# Autodesk Inventor assembly: 176-DP(D-229)(F,D-231-1)
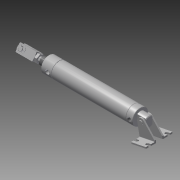
[picture p0: Inventor's stored thumbnail of the model, 180x180]
Saved by Autodesk Inventor 2014 (Build 180170000, 170)
## iProperties
Category: PARTsolutions
Company: BIMBA
Created: 2014-01-18
Part Number: 176-DP(D-229)(F,D-231-1)
Catalog Web Link: www.cadenas.de
Description: Original Line Standard Air Cylinders-
Vendor: BIMBA
Document SubType Name: Assembly
Designer: Andrew Toennies
Manufacturer: BIMBA
Mass: 1194.98 g
Surface Area: 947.453 cm^2
Volume: 152.227 cm^3
Density: 7.85 g/cm^3
PSOL_IDENT_0: {$CADENAS_DATA\23d-libs\bimba\bimba\bimba_imperial\bimba_full_line\original_line_cylinders\standard_
PSOL_IDENT_1: air_cylinders\standard_air_cylinder_asmtab.prj},330 {VTYP=3D},{STYP=ASSTAB},{NB=176-DP(D-229)(F,D-23
PSOL_IDENT_2: 1-1)},{LINA=176-DP},{NN=Original Line Standard Air Cylinders},{DATE=11.10.2013 11:47:29},{GEOMDATE=1
PSOL_IDENT_3: 7.04.2013 07:27:53},{VERSION=},{LINEID=80},{LINESUBID=-1},{WBVAR=STROKE,ACTING,MNT,DER,NR,BM,CO,OO,V
PSOL_IDENT_4: O,M,EE,EEL,K,Q,Y,G,T,B,H,SER,SR,NT,W,HL,STPT1,STPT2,STPT3,STPT4,MB,PB,PRC,TB,MN}  {NB=176-DP(D-229)(
PSOL_IDENT_5: F,D-231-1)},{LINA=176-DP},{KT=DUMMY},{PN=176-DP},{PNC=176-DP(D-229)(F,D-231-1)},{PNA=(D-229)(D-231-1
PSOL_IDENT_6: )},{DASH=-},{BORE1=1.50000000},{BORE=1 1/2\" (17)},{BOREPN=17},{STROKE=6.000},{STROKEALG=[0.011:50/0
PSOL_IDENT_7: .001]},{STROKE1=6.000},{ACTING=D},{ACTINGALG= '' , 'Single Acting (SA)' , 'R' , 'Reverse Single Acti
PSOL_IDENT_8: ng (SA)' , 'D' , 'Double Acting (SA)' },{ACTINGPN=D},{MNT=P},{MNTALG= '' , 'Front Nose Mounting (SA)'
PSOL_IDENT_9: , 'P' , 'Rear Pivot Mounting (SA)' , 'X' , 'Double End Mounting (SA)' , 'BF' , 'Front Block Mountin
PSOL_IDENT_10: g (SA)' , 'BR' , 'Rear Block Mounting for Vertical Positioning (SA)' , 'BFT' , 'Front Block Trunnion
PSOL_IDENT_11: Mounting (SA)' , 'BRT' , 'Rear Block Trunnion Mounting (SA)' },{TYPE=},{MNTPN=P},{DER=},{DERALG= ''
PSOL_IDENT_12: , 'N/A' },{NR=},{NRALG= '' , 'N/A' },{NRPN=},{BM=},{BMALG= '' , 'N/A' },{BMPN=},{CO=},{COALG= '' , '
PSOL_IDENT_13: N/A' },{OO=},{OOALG= '', 'N/A' },{OOPN=},{VO=Z},{VOALG= 'Z' , 'N/A' },{VOPN=},{OOVOPN=},{M=},{MALG= ''
PSOL_IDENT_14: , 'Without Magnet', 'M', 'With Magnet' },{EE=},{EEL=0.000},{EEMAX=44.0000},{EEALG= '', 'Without Extr
PSOL_IDENT_15: a Extension', 'EE', 'With Extra Extension' },{EELALG=0},{EEPN=},{EEPN1=0.000},{K=},{KALG= '', 'Stand
PSOL_IDENT_16: ard' , 'K' , 'Ports Rotated 90deg K' },{KPN=},{Q=},{QALG= '' , 'N/A' },{QPN=},{Y=},{YALG= '' , 'With
PSOL_IDENT_17: out Pivot Bushing' , 'Y' , 'With Pivot Bushing' },{YPN=},{YCON=},{F=},{FALG= '', 'Non-Coated (Standa
PSOL_IDENT_18: rd)', 'F', 'Molycoated' },{FPN=},{G=},{GPN=},{GPN99=},{T=},{TALG= '' , 'Standard -20° to 200°F (-29°
PSOL_IDENT_19: to 95°C)' , 'N' , 'Low Temperature' , 'V' , 'High Temperature' },{NPN=},{VPN=},{B=},{BALG= '', 'W/o
PSOL_IDENT_20: ut Bumpers' , 'B' , 'W/ Bumpers' },{BPN=},{H=},{HALG= '', 'N/A' },{HPN=},{SER=},{SERALG= '' , 'Witho
PSOL_IDENT_21: ut Spring Extend/Return' , 'JS' , 'With Spring Return' , 'JR' , 'With Spring Extend' },{SR=C},{SRALG=
PSOL_IDENT_22: 'C' , 'Standard Blackened Carbon Steel' , 'SR' , 'Stainless Steel [SR]' },{SRPN=},{SRCON=1},{NT=},{
PSOL_IDENT_23: NTPN=},{W=},{WALG= '' , 'Without Wiper' , 'W' , 'With Wiper' },{WPN=},{E=},{EALG= '' , 'Standard Sea
PSOL_IDENT_24: ls/Lube' , 'E' , 'Non-Lube Seals/Lube' },{EPN=},{HL=},{HLALG= '' , 'Without Low Pressure Hydraulic'
PSOL_IDENT_25: , 'HL' , 'With Low Pressure Hydraulic' },{ST=},{STALG= '' , 'N/A' },{STPT1=},{STPT1ALG= '' , 'N/A' }
PSOL_IDENT_26: ,{STPT2=},{STPT2ALG= '' , 'N/A' },{STPT3=},{STPT3ALG= '' , 'N/A' },{STPT4=},{STPT4ALG= '' , 'N/A' },
PSOL_IDENT_27: {STPN=},{MB=},{MBALG= '' , 'Without Mounting Bracket' , 'F,D-241' , 'D-241 (front)' },{MBPN=},{MBPNA
PSOL_IDENT_28: LL=D-241},{MBPNALLREAR=},{PB=D-229},{PBALG= '' , 'Without Pivot Bracket' , 'D-229' , 'D-229' },{PBPN=
PSOL_IDENT_29: (D-229)},{PBPNALL=D-229},{PRC=F,D-231-1},{PRCALG= '' , 'W/out Pivot Rod Clevis' , 'F,D-231-1' , 'D-2
PSOL_IDENT_30: 31-1 (front)' },{PRCPN=(F,D-231-1)},{PRCPNALL=D-231-1},{TB=},{TBALG= '' , 'N/A' },{TBPN=},{TBPNALL=}
PSOL_IDENT_31: ,{MN=},{MNALG= '' , 'Without Mounting Nut' , 'F,D-3556' , 'D-3556 (front)'},{MNPN=},{MNCONF=},{MNCON
PSOL_IDENT_32: R=},{TLEN=7.3025},{FRAC=45.3800},{RGCON=},{RGDACCON=R},{RHCON=P},{RHCON1=P},{RHCONON=1},{RHACCON=R},
PSOL_IDENT_33: {FNUTCON=0},{RNUTCON=0},{FNUTPN=D-3556},{RNUTPN=},{FNUTTRANS=0.0000},{RNUTTRANS=0.0000},{VHOLECON=0}
PSOL_IDENT_34: ,{A1=1.8750},{A1N=1.3120},{A1P=1.8750},{A1B=2.3750},{A4=0.2525},{A4N=0.5000},{A4P=0.2525},{A5=0.0400
PSOL_IDENT_35: },{A1H=1.75},{A1NH=0.6880},{A1PH=1.7500},{A1BH=1.3750},{A1SH=1.5000},{A2H=0.2500},{A2NH=0.2500},{LEN
PSOL_IDENT_36: GTH=4.3800},{LENGTH1=4.3800},{LENGTH2=4.4400},{MUL=6.0000},{MUL11=6.0000},{MUL22=16.14},{MUL33=10.14
PSOL_IDENT_37: 00},{MUL2=6.0000},{MUL211=6.0000},{MUL222=2.6900},{MUL233=1.6900},{SSS=12.0000},{RGLEN=1.6625},{RHLE
PSOL_IDENT_38: N=1.1650},{SSS1=7.0000},{A13=1.3750},{DIF=0.2500},{G5=0.0000},{ON=0},{SSADD=0.0000},{BADD=0.0000},{M
PSOL_IDENT_39: ADD=0.0000},{NVADD=0.0000},{TRACKL=7.0325},{TRACKCON=D-78527},{TRIMCON=0},{TRIMCON1=0},{PINCON=D-358
PSOL_IDENT_40: },{FSPACE=1.2186},{SPACE=0.2143},{TEXT=0.3750},{S1=1.7500},{D1=1.5800},{D1N=1.5565},{D1B=1.5565},{D1
PSOL_IDENT_41: P=1.5800},{FA=1.120},{RA=1.1200},{PPATH=standard_air_cylinder_asmtpl.prj},{MATALGHTML=<b>Standard Or
PSOL_IDENT_42: iginal Line:</b><dl><dt>Rod:</dt><dd>- Stainless Steel</dd><dd>&nbsp;&nbsp;(5/16 9/16 Bores)</dd><dd
PSOL_IDENT_43: >- High Strength Carbon Steel</dd><dd>&nbsp;&nbsp;(3/4 3 Bore)</dd><dd>- Stainless Steel</dd><dd>&nb
PSOL_IDENT_44: sp;&nbsp;(X style DXP/DX/DXDE)</dd><dt>Bearings:</dt><dd>- Sintered Bronze</dd><dt>Body:</dt><dd>- 3
PSOL_IDENT_45: 04 Stainless Steel</dd><dt>End Caps:</dt><dd>- Aluminum</dd><dt>Seals:</dt><dd>- Buna N</dd></dl>},{
PSOL_IDENT_46: ASSCFGPRA=17DP},{MBPNA=},{MNPNA=},{PRCPNA=(D-231-1)},{ASSOPTACC=STPT4},{A=10.38},{HADD=0.0000},{WFL=
PSOL_IDENT_47: 0.25},{QADD=0.000},{QADD1=0.190},{TEST=6.0000},{MNTB=},{STDNUTF=0},{STDNUTR=0}
CNS_NN: Original Line Standard Air Cylinders
CNS_NT: Standard Male Thread
CNS_NB: 176-DP(D-229)(F,D-231-1)
CNS_NBSYN: $PNC.
CNS_LINA: 176-DP
CNS_PN: 176-DP
CNS_PNC: 176-DP(D-229)(F,D-231-1)
CNS_PNA: (D-229)(D-231-1)
CNS_DASH: -
CNS_BORE1: 1.50000000
CNS_BORE: 1 1/2" [17]
CNS_BOREPN: 17
CNS_STROKE: 6.000
CNS_STROKEALG: [0.011:50/0.001]
CNS_STROKE1: 6.000
CNS_ACTING: Double [D]
CNS_ACTINGALG: '' , 'Single Acting (SA)' , 'R' , 'Reverse Single Acting (SA)' , 'D' , 'Double Acting (SA)'
CNS_ACTINGPN: D
CNS_MNT: Rear Pivot [P]
CNS_MNTALG: '' , 'Front Nose Mounting (SA)' , 'P' , 'Rear Pivot Mounting (SA)' , 'X' , 'Double End Mounting (SA)' , 'BF' , 'Front Block Mounting (SA)' , 'BR' , 'Rear Block Mounting for Vertical Positioning (SA)' , 'BFT' , 'Front Block Trunnion Mounting (SA)' , 'BRT' , 'Rear Block Trunnion Mounting (SA)'
CNS_MNTPN: P
CNS_DER: N/A
CNS_DERALG: '' , 'N/A'
CNS_NR: N/A
CNS_NRALG: '' , 'N/A'
CNS_BM: N/A
CNS_BMALG: '' , 'N/A'
CNS_CO: N/A
CNS_COALG: '' , 'N/A'
CNS_OO: N/A
CNS_OOALG: '', 'N/A'
CNS_VO: N/A
CNS_VOALG: 'Z' , 'N/A'
CNS_M: Without Magnet Piston
CNS_MALG: '', 'Without Magnet', 'M', 'With Magnet'
CNS_EE: Standard Rod Extension
CNS_EEL: 0.000
CNS_EEMAX: 44.0000
CNS_EEALG: '', 'Without Extra Extension', 'EE', 'With Extra Extension'
CNS_EELALG: 0
CNS_EEPN1: 0.000
CNS_K: Standard
CNS_KALG: '', 'Standard' , 'K' , 'Ports Rotated 90deg K'
CNS_Q: N/A
CNS_QALG: '' , 'N/A'
CNS_Y: Standard Pivot Style
CNS_YALG: '' , 'Without Pivot Bushing' , 'Y' , 'With Pivot Bushing'
CNS_FALG: '', 'Non-Coated (Standard)', 'F', 'Molycoated'
CNS_G: Standard Grease Lube
CNS_T: Standard -20° to 200°F (-29° to 95°C)
CNS_TALG: '' , 'Standard -20° to 200°F (-29° to 95°C)' , 'N' , 'Low Temperature' , 'V' , 'High Temperature'
CNS_B: Without Bumpers
CNS_BALG: '', 'W/out Bumpers' , 'B' , 'W/ Bumpers'
CNS_H: N/A
CNS_HALG: '', 'N/A'
CNS_SER: Without Failsafe Spring Extend/Return
CNS_SERALG: '' , 'Without Spring Extend/Return' , 'JS' , 'With Spring Return' , 'JR' , 'With Spring Extend'
CNS_SR: Standard Blackened Carbon Steel
CNS_SRALG: 'C' , 'Standard Blackened Carbon Steel' , 'SR' , 'Stainless Steel [SR]'
CNS_SRCON: 1
CNS_W: Without Wiper
CNS_WALG: '' , 'Without Wiper' , 'W' , 'With Wiper'
CNS_EALG: '' , 'Standard Seals/Lube' , 'E' , 'Non-Lube Seals/Lube'
CNS_HL: Standard 250 PSI Air
CNS_HLALG: '' , 'Without Low Pressure Hydraulic' , 'HL' , 'With Low Pressure Hydraulic'
CNS_STALG: '' , 'N/A'
CNS_STPT1: N/A
CNS_STPT1ALG: '' , 'N/A'
CNS_STPT2: N/A
CNS_STPT2ALG: '' , 'N/A'
CNS_STPT3: N/A
CNS_STPT3ALG: '' , 'N/A'
CNS_STPT4: N/A
CNS_STPT4ALG: '' , 'N/A'
CNS_MB: Without Mounting Bracket
CNS_MBALG: '' , 'Without Mounting Bracket' , 'F,D-241' , 'D-241 (front)'
CNS_MBPNALL: D-241
CNS_PB: D-229
CNS_PBALG: '' , 'Without Pivot Bracket' , 'D-229' , 'D-229'
CNS_PBPN: (D-229)
CNS_PBPNALL: D-229
CNS_PRC: D-231-1 (front)
CNS_PRCALG: '' , 'W/out Pivot Rod Clevis' , 'F,D-231-1' , 'D-231-1 (front)'
CNS_PRCPN: (F,D-231-1)
CNS_PRCPNALL: D-231-1
CNS_TB: N/A
CNS_TBALG: '' , 'N/A'
CNS_MN: Without Mounting Nut
CNS_MNALG: '' , 'Without Mounting Nut' , 'F,D-3556' , 'D-3556 (front)'
CNS_TLEN: 7.3025
CNS_FRAC: 45.3800
CNS_RGDACCON: R
CNS_RHCON: P
CNS_RHCON1: P
CNS_RHCONON: 1
CNS_RHACCON: R
CNS_FNUTCON: 0
CNS_RNUTCON: 0
CNS_FNUTPN: D-3556
CNS_FNUTTRANS: 0.0000
CNS_RNUTTRANS: 0.0000
CNS_VHOLECON: 0
CNS_A1: 1.8750
CNS_A1N: 1.3120
CNS_A1P: 1.8750
CNS_A1B: 2.3750
CNS_A4: 0.2525
CNS_A4N: 0.5000
CNS_A4P: 0.2525
CNS_A5: 0.0400
CNS_A1H: 1.750
CNS_A1NH: 0.6880
CNS_A1PH: 1.7500
CNS_A1BH: 1.3750
CNS_A1SH: 1.5000
CNS_A2H: 0.2500
CNS_A2NH: 0.2500
CNS_LENGTH: 4.3800
CNS_LENGTH1: 4.3800
CNS_LENGTH2: 4.4400
CNS_MUL: 6.0000
CNS_MUL11: 6.0000
CNS_MUL22: 16.140
CNS_MUL33: 10.1400
CNS_MUL2: 6.0000
CNS_MUL211: 6.0000
CNS_MUL222: 2.6900
CNS_MUL233: 1.6900
CNS_SSS: 12.0000
CNS_RGLEN: 1.6625
CNS_RHLEN: 1.1650
CNS_SSS1: 7.0000
CNS_A13: 1.3750
CNS_DIF: 0.2500
CNS_G5: 0.0000
CNS_ON: 0
CNS_SSADD: 0.0000
CNS_BADD: 0.0000
CNS_MADD: 0.0000
CNS_NVADD: 0.0000
CNS_TRACKL: 7.0325
CNS_TRACKCON: D-78527
CNS_TRIMCON: 0
CNS_TRIMCON1: 0
CNS_PINCON: D-358
CNS_FSPACE: 1.2186
CNS_SPACE: 0.2143
CNS_TEXT: 0.3750
CNS_S1: 1.7500
CNS_D1: 1.5800
CNS_D1N: 1.5565
CNS_D1B: 1.5565
CNS_D1P: 1.5800
CNS_FA: 1.120
CNS_RA: 1.1200
CNS_PPATH: standard_air_cylinder_asmtpl.prj
CNS_MATALGHTML: <b>Standard Original Line:</b><dl><dt>Rod:</dt><dd>- Stainless Steel</dd><dd>&nbsp;&nbsp;(5/16 9/16 Bores)</dd><dd>- High Strength Carbon Steel</dd><dd>&nbsp;&nbsp;(3/4 3 Bore)</dd><dd>- Stainless Steel</dd><dd>&nbsp;&nbsp;(X style DXP/DX/DXDE)</dd><dt>Bearings:</dt><dd>- Sintered Bronze</dd><dt>Body:</dt><dd>- 304 Stainless Steel</dd><dt>End Caps:</dt><dd>- Aluminum</dd><dt>Seals:</dt><dd>- Buna N</dd></dl>
CNS_ASSCFGPRA: 17DP
CNS_PRCPNA: (D-231-1)
CNS_ASSOPTACC: STPT4
CNS_A: 10.38
CNS_HADD: 0.0000
CNS_WFL: 0.250
CNS_QADD: 0.000
CNS_QADD1: 0.190
CNS_TEST: 6.0000
CNS_STDNUTF: 0
CNS_STDNUTR: 0
SUPPLIER: BIMBA
ARTICLENO: 176-DP(D-229)(F,D-231-1)
BOMINFO: 176-DP
CREATOR: CADENAS GmbH
Title: 176-DP
Author: Cadenas PARTsolutions
## Documents named in this file (15)
- C:\Users\Andrew Toennies\Documents\GitHub\2014buildCAD\New Shooter\1.5 in bore 6 in stroke cylinder - BIMBA\176-DP(D-229)(F,D-231-1).iam
- C:\Users\Andrew Toennies\Documents\GitHub\2014buildCAD\New Shooter\1.5 in bore 6 in stroke cylinder - BIMBA\176-DPC(D-229)(F,D-231-1)0000_0_dummy.ipt
- C:\Users\Andrew Toennies\Documents\GitHub\2014buildCAD\New Shooter\1.5 in bore 6 in stroke cylinder - BIMBA\17R000-0_rod_guide.ipt
- C:\Users\Andrew Toennies\Documents\GitHub\2014buildCAD\New Shooter\1.5 in bore 6 in stroke cylinder - BIMBA\17R-7_30250C.ipt
- C:\Users\Andrew Toennies\Documents\GitHub\2014buildCAD\New Shooter\1.5 in bore 6 in stroke cylinder - BIMBA\17P0000_rear_head.ipt
- C:\Users\Andrew Toennies\Documents\GitHub\2014buildCAD\New Shooter\1.5 in bore 6 in stroke cylinder - BIMBA\D-358.ipt
- C:\Users\Andrew Toennies\Documents\GitHub\2014buildCAD\New Shooter\1.5 in bore 6 in stroke cylinder - BIMBA\D-229-dummy.ipt
- C:\Users\Andrew Toennies\Documents\GitHub\2014buildCAD\New Shooter\1.5 in bore 6 in stroke cylinder - BIMBA\D-9969.ipt
- C:\Users\Andrew Toennies\Documents\GitHub\2014buildCAD\New Shooter\1.5 in bore 6 in stroke cylinder - BIMBA\D-14826.ipt
- C:\Users\Andrew Toennies\Documents\GitHub\2014buildCAD\New Shooter\1.5 in bore 6 in stroke cylinder - BIMBA\C-176-DP0_rod.ipt
- C:\Users\Andrew Toennies\Documents\GitHub\2014buildCAD\New Shooter\1.5 in bore 6 in stroke cylinder - BIMBA\D-231-1-dummy.ipt
- C:\Users\Andrew Toennies\Documents\GitHub\2014buildCAD\New Shooter\1.5 in bore 6 in stroke cylinder - BIMBA\D-14053.ipt
- C:\Users\Andrew Toennies\Documents\GitHub\2014buildCAD\New Shooter\1.5 in bore 6 in stroke cylinder - BIMBA\D-8383.ipt
- C:\Users\Andrew Toennies\Documents\GitHub\2014buildCAD\New Shooter\1.5 in bore 6 in stroke cylinder - BIMBA\D-5867.ipt
- C:\Users\Andrew Toennies\Documents\GitHub\2014buildCAD\New Shooter\1.5 in bore 6 in stroke cylinder - BIMBA\D-154.ipt
## Components (15 placed, 14 different names)
1. 176-DPC(D-229)(F,D-231-1)0000_0_dummy:1 — dummy_XY@1 <-> rod_guide_XY@2, dummy_Z@1 <-> rod_guide_Z@2, dummy_YZ@1 <-> rod_guide_YZ@2
2. 17R000-0_rod_guide:1 — dummy_XY@1 <-> rod_guide_XY@2, dummy_Z@1 <-> rod_guide_Z@2, dummy_YZ@1 <-> rod_guide_YZ@2, to_tube_XY@2 <-> tube_front_XY@3, to_tube_Z@2 <-> tube_front_Z@3, to_tube_YZ@2 <-> tube_front_YZ@3, to_rod_XY@2 <-> rod_cp_XY@9, to_rod_Z@2 <-> rod_cp_Z@9
3. 17R-7_30250C:1 — to_tube_XY@2 <-> tube_front_XY@3, to_tube_Z@2 <-> tube_front_Z@3, to_tube_YZ@2 <-> tube_front_YZ@3, tube_rear_XY@3 <-> to_tube_XY@4, tube_rear_Z@3 <-> to_tube_Z@4, tube_rear_YZ@3 <-> to_tube_YZ@4
4. 17P0000_rear_head:1 — tube_rear_XY@3 <-> to_tube_XY@4, tube_rear_Z@3 <-> to_tube_Z@4, tube_rear_YZ@3 <-> to_tube_YZ@4, to_pin_XY@4 <-> pin_XY@5, to_pin_Z@4 <-> pin_Z@5, to_pin_YZ@4 <-> pin_YZ@5, to_pin_XY@4 <-> to_cyl_XY@6, to_pin_Z@4 <-> to_cyl_Z@6
5. D-358:1 — to_pin_XY@4 <-> pin_XY@5, to_pin_Z@4 <-> pin_Z@5, to_pin_YZ@4 <-> pin_YZ@5
6. D-229-dummy:1 — to_pin_XY@4 <-> to_cyl_XY@6, to_pin_Z@4 <-> to_cyl_Z@6, to_l_XY@6 <-> to_dummy_L_XY@7, to_l_Z@6 <-> to_dummy_L_Z@7, to_l_YZ@6 <-> to_dummy_L_YZ@7, to_r_XY@6 <-> to_dummy_R_XY@8, to_r_Z@6 <-> to_dummy_R_Z@8, to_r_YZ@6 <-> to_dummy_R_YZ@8
7. D-9969:1 — to_l_XY@6 <-> to_dummy_L_XY@7, to_l_Z@6 <-> to_dummy_L_Z@7, to_l_YZ@6 <-> to_dummy_L_YZ@7
8. D-14826:1 — to_r_XY@6 <-> to_dummy_R_XY@8, to_r_Z@6 <-> to_dummy_R_Z@8, to_r_YZ@6 <-> to_dummy_R_YZ@8
9. C-176-DP0_rod:1 — to_rod_XY@2 <-> rod_cp_XY@9, to_rod_Z@2 <-> rod_cp_Z@9, to_rod_clevis_XY@9 <-> to_cyl_XY@10, to_rod_clevis_Z@9 <-> to_cyl_Z@10, to_rod_clevis_YZ@9 <-> to_cyl_YZ@10
10. D-231-1-dummy:1 — to_rod_clevis_XY@9 <-> to_cyl_XY@10, to_rod_clevis_Z@9 <-> to_cyl_Z@10, to_rod_clevis_YZ@9 <-> to_cyl_YZ@10, dummy_XY@10 <-> dummy_XY@11, dummy_Z@10 <-> dummy_Z@11, dummy_YZ@10 <-> dummy_YZ@11
11. D-14053:1 — dummy_XY@10 <-> dummy_XY@11, dummy_Z@10 <-> dummy_Z@11, dummy_YZ@10 <-> dummy_YZ@11, rod_clevis_body_XY@11 <-> pin_XY@12, rod_clevis_body_Z@11 <-> pin_Z@12, piston_rod_clevis_XY@11 <-> NUT_XY@15, piston_rod_clevis_Z@11 <-> NUT_Z@15
12. D-8383:1 — rod_clevis_body_XY@11 <-> pin_XY@12, rod_clevis_body_Z@11 <-> pin_Z@12, rr1_XY@12 <-> RR_XY@13, rr1_Z@12 <-> RR_Z@13, rr2_XY@12 <-> RR_XY@14, rr2_Z@12 <-> RR_Z@14
13. D-5867:1 — rr1_XY@12 <-> RR_XY@13, rr1_Z@12 <-> RR_Z@13
14. D-5867:2 — rr2_XY@12 <-> RR_XY@14, rr2_Z@12 <-> RR_Z@14
15. D-154:1 — piston_rod_clevis_XY@11 <-> NUT_XY@15, piston_rod_clevis_Z@11 <-> NUT_Z@15
## Relationships (36: Mate 20, Flush 8, Angle 8)
- dummy_XY@1 <-> rod_guide_XY@2 [Flush]: 176-DPC(D-229)(F,D-231-1)0000_0_dummy:1 ↔ 17R000-0_rod_guide:1
- dummy_Z@1 <-> rod_guide_Z@2 [Mate]: 176-DPC(D-229)(F,D-231-1)0000_0_dummy:1 ↔ 17R000-0_rod_guide:1
- dummy_YZ@1 <-> rod_guide_YZ@2 [Angle] (0 deg): 176-DPC(D-229)(F,D-231-1)0000_0_dummy:1 ↔ 17R000-0_rod_guide:1
- to_tube_XY@2 <-> tube_front_XY@3 [Flush]: 17R000-0_rod_guide:1 ↔ 17R-7_30250C:1
- to_tube_Z@2 <-> tube_front_Z@3 [Mate]: 17R000-0_rod_guide:1 ↔ 17R-7_30250C:1
- to_tube_YZ@2 <-> tube_front_YZ@3 [Angle] (0 deg): 17R000-0_rod_guide:1 ↔ 17R-7_30250C:1
- tube_rear_XY@3 <-> to_tube_XY@4 [Flush]: 17R-7_30250C:1 ↔ 17P0000_rear_head:1
- tube_rear_Z@3 <-> to_tube_Z@4 [Mate]: 17R-7_30250C:1 ↔ 17P0000_rear_head:1
- tube_rear_YZ@3 <-> to_tube_YZ@4 [Angle] (0 deg): 17R-7_30250C:1 ↔ 17P0000_rear_head:1
- to_pin_XY@4 <-> pin_XY@5 [Mate]: 17P0000_rear_head:1 ↔ D-358:1
- to_pin_Z@4 <-> pin_Z@5 [Mate]: 17P0000_rear_head:1 ↔ D-358:1
- to_pin_YZ@4 <-> pin_YZ@5 [Angle] (0 deg): 17P0000_rear_head:1 ↔ D-358:1
- to_pin_XY@4 <-> to_cyl_XY@6 [Flush]: 17P0000_rear_head:1 ↔ D-229-dummy:1
- to_pin_Z@4 <-> to_cyl_Z@6 [Mate]: 17P0000_rear_head:1 ↔ D-229-dummy:1
- to_l_XY@6 <-> to_dummy_L_XY@7 [Flush]: D-229-dummy:1 ↔ D-9969:1
- to_l_Z@6 <-> to_dummy_L_Z@7 [Mate]: D-229-dummy:1 ↔ D-9969:1
- to_l_YZ@6 <-> to_dummy_L_YZ@7 [Angle] (0 deg): D-229-dummy:1 ↔ D-9969:1
- to_r_XY@6 <-> to_dummy_R_XY@8 [Flush]: D-229-dummy:1 ↔ D-14826:1
- to_r_Z@6 <-> to_dummy_R_Z@8 [Mate]: D-229-dummy:1 ↔ D-14826:1
- to_r_YZ@6 <-> to_dummy_R_YZ@8 [Angle] (0 deg): D-229-dummy:1 ↔ D-14826:1
- to_rod_XY@2 <-> rod_cp_XY@9 [Flush]: 17R000-0_rod_guide:1 ↔ C-176-DP0_rod:1
- to_rod_Z@2 <-> rod_cp_Z@9 [Mate]: 17R000-0_rod_guide:1 ↔ C-176-DP0_rod:1
- to_rod_clevis_XY@9 <-> to_cyl_XY@10 [Flush]: C-176-DP0_rod:1 ↔ D-231-1-dummy:1
- to_rod_clevis_Z@9 <-> to_cyl_Z@10 [Mate]: C-176-DP0_rod:1 ↔ D-231-1-dummy:1
- to_rod_clevis_YZ@9 <-> to_cyl_YZ@10 [Angle] (0 deg): C-176-DP0_rod:1 ↔ D-231-1-dummy:1
- dummy_XY@10 <-> dummy_XY@11 [Mate]: D-231-1-dummy:1 ↔ D-14053:1
- dummy_Z@10 <-> dummy_Z@11 [Mate]: D-231-1-dummy:1 ↔ D-14053:1
- dummy_YZ@10 <-> dummy_YZ@11 [Angle] (0 deg): D-231-1-dummy:1 ↔ D-14053:1
- rod_clevis_body_XY@11 <-> pin_XY@12 [Mate]: D-14053:1 ↔ D-8383:1
- rod_clevis_body_Z@11 <-> pin_Z@12 [Mate]: D-14053:1 ↔ D-8383:1
- rr1_XY@12 <-> RR_XY@13 [Mate]: D-8383:1 ↔ D-5867:1
- rr1_Z@12 <-> RR_Z@13 [Mate]: D-8383:1 ↔ D-5867:1
- rr2_XY@12 <-> RR_XY@14 [Mate]: D-8383:1 ↔ D-5867:2
- rr2_Z@12 <-> RR_Z@14 [Mate]: D-8383:1 ↔ D-5867:2
- piston_rod_clevis_XY@11 <-> NUT_XY@15 [Mate]: D-14053:1 ↔ D-154:1
- piston_rod_clevis_Z@11 <-> NUT_Z@15 [Mate]: D-14053:1 ↔ D-154:1
